# Autodesk Inventor assembly: s-assy-spacer3
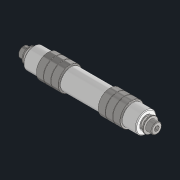
[picture p0: Inventor's stored thumbnail of the model, 180x180]
Saved by Autodesk Inventor 2021 (Build 250183000, 183)
## iProperties
Created: 2021-07-17
Part Number: s-assy-spacer3
Document SubType Name: Assembly
Designer: yuta0
Author: yuta0
## Documents named in this file (7)
- C:\Users\yuta0\Desktop\catchrobo_robot\s-assy-spacer3.iam
- C:\Users\yuta0\Desktop\catchrobo_robot\B688ZZ.ipt
- C:\Users\yuta0\Desktop\catchrobo_robot\base21.ipt
- C:\Users\yuta0\Desktop\catchrobo_robot\base22.ipt
- C:\Users\yuta0\Desktop\catchrobo_robot\SFHRW8-76-M4-N4.ipt
- C:\Users\yuta0\Desktop\lab\nicebot\CB4-10.ipt
- C:\Users\yuta0\Desktop\catchrobo_robot\WSJ-STN-M4.ipt
## Components (14 placed, 6 different names)
1. SFHRW8-76-M4-N4:1 — メイト:33, メイト:34, メイト:35, メイト:36
2. base22:1 — メイト:30, メイト:31
3. base21:3 — メイト:32
4. base21:4 — メイト:29
5. CB4-10:1 — メイト:33, メイト:36, メイト:39, メイト:40
6. CB4-10:2 — メイト:34, メイト:35, メイト:37, メイト:38
7. WSJ-STN-M4:1 — メイト:37, メイト:38
8. WSJ-STN-M4:2 — メイト:39, メイト:40
9. B688ZZ:2 — メイト:31
10. B688ZZ:5 — メイト:29
11. B688ZZ:6
12. B688ZZ:7
13. B688ZZ:8 — メイト:32
14. B688ZZ:9 — メイト:30
## Component patterns: (3 elements, first: B688ZZ:2 + B688ZZ:5)
## Relationships (18: Mate 17, Flush 1)
- [Mate]: SFHRW8-76-M4-N4:1 ↔ base22:1
- [Mate]: SFHRW8-76-M4-N4:1 ↔ base21:3
- [Mate]: SFHRW8-76-M4-N4:1 ↔ base21:4
- [Mate]: SFHRW8-76-M4-N4:1 ↔ B688ZZ:5
- [Mate]: SFHRW8-76-M4-N4:1 ↔ B688ZZ:2
- [Flush]: SFHRW8-76-M4-N4:1 ↔ base21:4
- メイト:29 [Mate]: base21:4 ↔ B688ZZ:5
- メイト:30 [Mate]: base22:1 ↔ B688ZZ:9
- メイト:31 [Mate]: base22:1 ↔ B688ZZ:2
- メイト:32 [Mate]: base21:3 ↔ B688ZZ:8
- メイト:33 [Mate]: SFHRW8-76-M4-N4:1 ↔ CB4-10:1
- メイト:34 [Mate]: SFHRW8-76-M4-N4:1 ↔ CB4-10:2
- メイト:35 [Mate] (3 mm): SFHRW8-76-M4-N4:1 ↔ CB4-10:2
- メイト:36 [Mate] (3 mm): SFHRW8-76-M4-N4:1 ↔ CB4-10:1
- メイト:37 [Mate]: CB4-10:2 ↔ WSJ-STN-M4:1
- メイト:38 [Mate]: CB4-10:2 ↔ WSJ-STN-M4:1
- メイト:39 [Mate]: CB4-10:1 ↔ WSJ-STN-M4:2
- メイト:40 [Mate]: CB4-10:1 ↔ WSJ-STN-M4:2
